# Autodesk Inventor assembly: Display_Unit
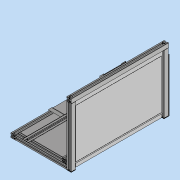
[picture p0: Inventor's stored thumbnail of the model, 180x180]
Saved by Autodesk Inventor 2020 (Build 240168000, 168)
## iProperties
Created: 2021-04-28
Part Number: Display_Unit
Document SubType Name: Assembly
Designer: ken113
Author: ken113
## Documents named in this file (11)
- C:\Users\lvglv\Documents\GitHub\Eto_Project\Hardware\Asem\Display_Unit.iam
- C:\Users\lvglv\Documents\GitHub\Eto_Project\Hardware\Parts\Display\Display.ipt
- C:\Users\lvglv\Documents\GitHub\Eto_Project\Hardware\Parts\MISUMI\NFS5-2020-437_Autodesk_Inventor_2020_20210429\NFS5-2020-437.ipt
- C:\Users\lvglv\Documents\GitHub\Eto_Project\Hardware\Parts\MISUMI\HFBL5-2020-200_Autodesk_Inventor_2020_20210429\AIS2020\HFBL5-2020-200_.ipt
- C:\Users\lvglv\Documents\GitHub\Eto_Project\Hardware\Parts\Meviy\Display_Angle.ipt
- C:\Users\lvglv\Documents\GitHub\Eto_Project\Hardware\Parts\MISUMI\NFSF5-2020-231_Autodesk_Inventor_2020_20210429\NFSF5-2020-231.ipt
- C:\Users\lvglv\Documents\GitHub\Eto_Project\Hardware\Parts\MISUMI\NFSF5-2020-263.5_Autodesk_Inventor_2020_20210429\NFSF5-2020-263_5.ipt
- C:\Users\lvglv\Documents\GitHub\Eto_Project\Hardware\Parts\MISUMI\HFC5-2020-B_Autodesk_Inventor_2020_20210429\HFC5-2020-B.ipt
- C:\Users\lvglv\Documents\GitHub\Eto_Project\Hardware\Parts\MISUMI\NFSF5-2020-437-Z6-YA10-YB427_Autodesk_Inventor_2020_20210429\NFSF5-2020-437-Z6-YA10-YB427.ipt
- C:\Users\lvglv\Documents\GitHub\Eto_Project\Hardware\Parts\Meviy\Display_Angle_B.ipt
- C:\Users\lvglv\Documents\GitHub\Eto_Project\Hardware\Parts\Meviy\Display_CCM_Mount.ipt
## Components (16 placed, 10 different names)
1. HFBL5-2020-200_:1 — メイト:34, フラッシュ:36
2. HFBL5-2020-200_:2 — メイト:33, フラッシュ:35
3. Display_Angle:1 — 挿入:1, 挿入:2
4. Display:3 — メイト:25, フラッシュ:23, フラッシュ:24, 挿入:1, 挿入:2
5. NFSF5-2020-231:1 — フラッシュ:29, メイト:28, メイト:30, フラッシュ:32, メイト:33, フラッシュ:35, フラッシュ:39, フラッシュ:40
6. NFSF5-2020-231:2 — メイト:29, フラッシュ:30, フラッシュ:31, メイト:31, メイト:34
7. Display:4 — メイト:25, フラッシュ:23, フラッシュ:24, 挿入:3, 挿入:4
8. NFSF5-2020-263_5:1 — メイト:26, フラッシュ:25, フラッシュ:26, メイト:28, メイト:32, フラッシュ:33, フラッシュ:34, メイト:37, フラッシュ:38, フラッシュ:40
9. NFSF5-2020-263_5:2 — メイト:27, フラッシュ:27, フラッシュ:28, メイト:29, フラッシュ:30, フラッシュ:36
10. HFC5-2020-B:1 — メイト:26, フラッシュ:25, フラッシュ:26, フラッシュ:29
11. HFC5-2020-B:2 — メイト:27, フラッシュ:27, フラッシュ:28, フラッシュ:31
12. NFSF5-2020-437-Z6-YA10-YB427:1 — メイト:30, フラッシュ:32, メイト:31
13. NFSF5-2020-437-Z6-YA10-YB427:2 — メイト:32, フラッシュ:33, フラッシュ:34
14. NFS5-2020-437:1
15. Display_Angle_B:1 — 挿入:3, 挿入:4
16. Display_CCM_Mount:1 — メイト:37, フラッシュ:38, フラッシュ:39
## Relationships (41: Flush 22, Mate 15, Insert 4)
- [Mate] (1 mm): Display:3 ↔ NFSF5-2020-231:1
- [Flush]: Display:3 ↔ NFSF5-2020-231:1
- [Flush]: NFSF5-2020-231:1 ↔ NFSF5-2020-231:2
- [Mate] (1 mm): Display:3 ↔ NFSF5-2020-231:2
- [Flush]: NFSF5-2020-231:1 ↔ NFSF5-2020-231:2
- [Flush] (1 mm): Display:3 ↔ NFSF5-2020-231:1
- メイト:25 [Mate]: Display:3 ↔ Display:4
- フラッシュ:23 [Flush]: Display:3 ↔ Display:4
- フラッシュ:24 [Flush]: Display:3 ↔ Display:4
- メイト:26 [Mate]: NFSF5-2020-263_5:1 ↔ HFC5-2020-B:1
- フラッシュ:25 [Flush]: NFSF5-2020-263_5:1 ↔ HFC5-2020-B:1
- フラッシュ:26 [Flush]: NFSF5-2020-263_5:1 ↔ HFC5-2020-B:1
- メイト:27 [Mate]: NFSF5-2020-263_5:2 ↔ HFC5-2020-B:2
- フラッシュ:27 [Flush]: NFSF5-2020-263_5:2 ↔ HFC5-2020-B:2
- フラッシュ:28 [Flush]: NFSF5-2020-263_5:2 ↔ HFC5-2020-B:2
- フラッシュ:29 [Flush]: NFSF5-2020-231:1 ↔ HFC5-2020-B:1
- メイト:28 [Mate]: NFSF5-2020-231:1 ↔ NFSF5-2020-263_5:1
- メイト:29 [Mate]: NFSF5-2020-231:2 ↔ NFSF5-2020-263_5:2
- フラッシュ:30 [Flush]: NFSF5-2020-231:2 ↔ NFSF5-2020-263_5:2
- フラッシュ:31 [Flush]: NFSF5-2020-231:2 ↔ HFC5-2020-B:2
- メイト:30 [Mate]: NFSF5-2020-231:1 ↔ NFSF5-2020-437-Z6-YA10-YB427:1
- フラッシュ:32 [Flush]: NFSF5-2020-231:1 ↔ NFSF5-2020-437-Z6-YA10-YB427:1
- メイト:31 [Mate]: NFSF5-2020-231:2 ↔ NFSF5-2020-437-Z6-YA10-YB427:1
- メイト:32 [Mate]: NFSF5-2020-263_5:1 ↔ NFSF5-2020-437-Z6-YA10-YB427:2
- フラッシュ:33 [Flush]: NFSF5-2020-263_5:1 ↔ NFSF5-2020-437-Z6-YA10-YB427:2
- フラッシュ:34 [Flush]: NFSF5-2020-263_5:1 ↔ NFSF5-2020-437-Z6-YA10-YB427:2
- メイト:33 [Mate]: HFBL5-2020-200_:2 ↔ NFSF5-2020-231:1
- フラッシュ:35 [Flush]: HFBL5-2020-200_:2 ↔ NFSF5-2020-231:1
- メイト:34 [Mate]: HFBL5-2020-200_:1 ↔ NFSF5-2020-231:2
- フラッシュ:36 [Flush]: HFBL5-2020-200_:1 ↔ NFSF5-2020-263_5:2
- [Flush]: NFSF5-2020-231:1 ↔ NFS5-2020-437:1
- [Mate]: NFSF5-2020-263_5:1 ↔ NFS5-2020-437:1
- [Mate]: NFSF5-2020-231:1 ↔ NFS5-2020-437:1
- 挿入:1 [Insert]: Display_Angle:1 ↔ Display:3
- 挿入:2 [Insert]: Display_Angle:1 ↔ Display:3
- 挿入:3 [Insert]: Display:4 ↔ Display_Angle_B:1
- 挿入:4 [Insert]: Display:4 ↔ Display_Angle_B:1
- メイト:37 [Mate]: NFSF5-2020-263_5:1 ↔ Display_CCM_Mount:1
- フラッシュ:38 [Flush]: NFSF5-2020-263_5:1 ↔ Display_CCM_Mount:1
- フラッシュ:39 [Flush]: NFSF5-2020-231:1 ↔ Display_CCM_Mount:1
- フラッシュ:40 [Flush]: NFSF5-2020-231:1 ↔ NFSF5-2020-263_5:1
